# Autodesk Inventor assembly: Main
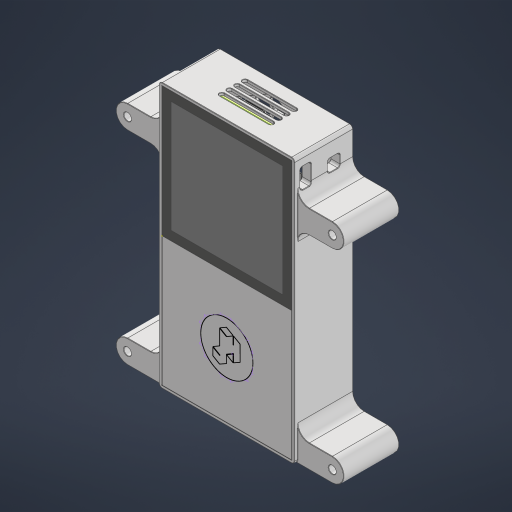
[picture p0: Inventor's stored thumbnail of the model, 512x512]
Saved by Autodesk Inventor 2023 (Build 270158000, 158)
## iProperties
Created: 2023-12-03
Part Number: Main
Document SubType Name: Assembly
Designer: FizzyApple12
Author: FizzyApple12
## Documents named in this file (9)
- C:\Users\FizzyApple12\Desktop\PurdueHackersDoorOpener\CAD\Main.iam
- C:\Users\FizzyApple12\Desktop\PurdueHackersDoorOpener\CAD\OTS\Hiletgo_PN532_module\PN532_NFC_Assembly.iam
- C:\Users\FizzyApple12\Desktop\PurdueHackersDoorOpener\CAD\OTS\Waveshare_4inch_LCD\4inch-hdmi-lcd_c.iam
- C:\Users\FizzyApple12\Desktop\PurdueHackersDoorOpener\CAD\PrimaryCase.ipt
- C:\Users\FizzyApple12\Desktop\PurdueHackersDoorOpener\CAD\OTS\Raspberry_Pi_3\raspberry_pi_3_b_plus.iam
- C:\Users\FizzyApple12\Desktop\PurdueHackersDoorOpener\CAD\ScanCover.ipt
- C:\Users\FizzyApple12\Desktop\PurdueHackersDoorOpener\CAD\OTS\Adafruit_Neopixel_Stick\NeoPixel Stick.iam
- C:\Users\FizzyApple12\Desktop\PurdueHackersDoorOpener\CAD\DoorButtonMount.ipt
- C:\Users\FizzyApple12\Desktop\PurdueHackersDoorOpener\CAD\ScanCoverMount.ipt
## Components (9 placed, 8 different names)
1. PN532_NFC_Assembly:1 [sub-assembly] — Flush:3, Mate:11, Mate:12
2. 4inch-hdmi-lcd_c:1 [sub-assembly] — Mate:5, Mate:6, Angle:1, Flush:1, Mate:7, Mate:8
3. PrimaryCase:1 — Flush:1, Mate:7, Mate:8, Mate:9, Flush:2, Mate:10, Flush:3, Mate:11, Mate:12, Mate:14, Mate:15, Mate:16, Mate:17, Mate:18, Mate:19, Mate:20, Mate:21, Mate:22
4. raspberry_pi_3_b_plus:1 [sub-assembly] — Mate:5, Mate:6, Angle:1
5. ScanCover:1 — Mate:9, Flush:2, Mate:10
6. NeoPixel Stick:1 [sub-assembly] — Mate:15, Mate:16, Mate:17
7. NeoPixel Stick:2 [sub-assembly] — Mate:14, Mate:18, Mate:19
8. DoorButtonMount:1
9. ScanCoverMount:1 — Mate:20, Mate:21, Mate:22
## Relationships (21: Mate 17, Flush 3, Angle 1)
- Mate:5: 4inch-hdmi-lcd_c:1 ↔ raspberry_pi_3_b_plus:1
- Mate:6: 4inch-hdmi-lcd_c:1 ↔ raspberry_pi_3_b_plus:1
- Angle:1 (0 deg): 4inch-hdmi-lcd_c:1 ↔ raspberry_pi_3_b_plus:1
- Flush:1: 4inch-hdmi-lcd_c:1 ↔ PrimaryCase:1
- Mate:7: 4inch-hdmi-lcd_c:1 ↔ PrimaryCase:1
- Mate:8: 4inch-hdmi-lcd_c:1 ↔ PrimaryCase:1
- Mate:9: PrimaryCase:1 ↔ ScanCover:1
- Flush:2: PrimaryCase:1 ↔ ScanCover:1
- Mate:10: PrimaryCase:1 ↔ ScanCover:1
- Flush:3 (-3 mm): PN532_NFC_Assembly:1 ↔ PrimaryCase:1
- Mate:11: PN532_NFC_Assembly:1 ↔ PrimaryCase:1
- Mate:12: PN532_NFC_Assembly:1 ↔ PrimaryCase:1
- Mate:14: PrimaryCase:1 ↔ NeoPixel Stick:2
- Mate:15: PrimaryCase:1 ↔ NeoPixel Stick:1
- Mate:16: PrimaryCase:1 ↔ NeoPixel Stick:1
- Mate:17: PrimaryCase:1 ↔ NeoPixel Stick:1
- Mate:18: PrimaryCase:1 ↔ NeoPixel Stick:2
- Mate:19: PrimaryCase:1 ↔ NeoPixel Stick:2
- Mate:20: PrimaryCase:1 ↔ ScanCoverMount:1
- Mate:21: PrimaryCase:1 ↔ ScanCoverMount:1
- Mate:22: PrimaryCase:1 ↔ ScanCoverMount:1
